# Autodesk Inventor assembly: LR_05
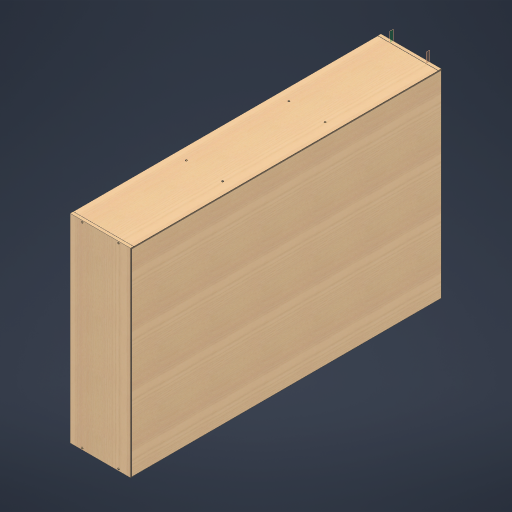
[picture p0: Inventor's stored thumbnail of the model, 512x512]
Saved by Autodesk Inventor 2024.3 (Build 283343000, 343)
## iProperties
Created: 2013-04-03
Part Number: LR_05
Document SubType Name: Assembly
Designer: User
Description: Rack
Author: User
## Documents named in this file (15)
- C:\W4INV 2024 Design\PROJECTS\Living Room\Rack\LR_05.iam
- C:\W4INV 2024 Design\PROJECTS\Samples\Living Room\Rack\LR_0502.ipt
- C:\W4INV 2024 Design\PROJECTS\Samples\Living Room\Rack\LR_0503.ipt
- C:\W4INV 2024 Design\PROJECTS\Samples\Living Room\Rack\LR_0508.ipt
- C:\W4INV 2024 Design\PROJECTS\Samples\Living Room\Rack\LR_0501.ipt
- C:\W4INV 2024 Design\PROJECTS\Samples\Living Room\Rack\LR_0506.ipt
- C:\W4INV 2024 Design\PROJECTS\Samples\Living Room\Rack\LR_0507.ipt
- C:\W4INV 2024 Design\PROJECTS\Samples\Living Room\Rack\LR_0504.ipt
- C:\W4INV 2024 Design\PROJECTS\Samples\Living Room\Rack\LR_0505.ipt
- C:\W4INV 2024 Design\PROJECTS\Samples\Living Room\Rack\SkeletonLR_0500.ipt
- G:\DESIGN\W4I 2014 EN\2013 COMPONENTS LIBRARY\01 CONNECTORS\01 CONFIRMAT\CONFIRMAT & HOLE & CAP.iam
- C:\W4INV 2023 Design\LIBRARY\Holders\Shelf holder D5.ipt
- C:\W4INV 2024 Design\_LIBRARY\Holders\Shelf holder D5\Shelf support D5 L16 HOL 3 CAP ON.ipt
- C:\W4INV 2024 Design\_LIBRARY\Fixed joints\Confirmat\CONFIRMAT\Confirmat L50 & Cap D10 NB T18 PB T 18.ipt
- C:\W4INV 2023 Design\LIBRARY\Fixed joints\Confirmat\CONFIRMAT.ipt
## Components (53 placed, 10 different names)
1. LR_0502-Right Side:2 — Nestled Board Plane:2, Nestled Board Plane:4, Nestled Board Plane:6, Nestled Board Plane:8
2. LR_0503-Left Side:2 — Flush:1, Flush:2, Mate:30, Mate:36, Nestled Board Plane:1, Nestled Board Plane:3, Nestled Board Plane:5, Nestled Board Plane:7
3. LR_0508-Top:2 — Pillar Board Side Plane:1, Pillar Board Side Plane:2, Pillar Board Side Plane:5, Pillar Board Side Plane:6, Nestled Board Plane:9, Nestled Board Plane:11, Nestled Board Plane:13, Nestled Board Plane:15
4. LR_0501-Bottom:2 — Pillar Board Side Plane:3, Pillar Board Side Plane:4, Pillar Board Side Plane:7, Pillar Board Side Plane:8, Nestled Board Plane:10, Nestled Board Plane:12, Nestled Board Plane:14, Nestled Board Plane:16
5. LR_0506-Vertical partition Left:2 — Mate:33, Mate:39, Pillar Board Side Plane:9, Pillar Board Side Plane:10, Pillar Board Side Plane:13, Pillar Board Side Plane:14
6. LR_0507-Vertical partition Right:2 — Pillar Board Side Plane:11, Pillar Board Side Plane:12, Pillar Board Side Plane:15, Pillar Board Side Plane:16
7. LR_0505-Back:2
8. Confirmat L50 & Cap D10 NB T18 PB T 18:1 — Axis Plane:1, Pillar Board Side Plane:1, Nestled Board Plane:1
9. Confirmat L50 & Cap D10 NB T18 PB T 18:2 — Axis Plane:2, Pillar Board Side Plane:2, Nestled Board Plane:2
10. Confirmat L50 & Cap D10 NB T18 PB T 18:3 — Axis Plane:3, Pillar Board Side Plane:3, Nestled Board Plane:3
11. Confirmat L50 & Cap D10 NB T18 PB T 18:4 — Axis Plane:4, Pillar Board Side Plane:4, Nestled Board Plane:4
12. Confirmat L50 & Cap D10 NB T18 PB T 18:5 — Axis Plane:5, Pillar Board Side Plane:5, Nestled Board Plane:5
13. Confirmat L50 & Cap D10 NB T18 PB T 18:6 — Axis Plane:6, Pillar Board Side Plane:6, Nestled Board Plane:6
14. Confirmat L50 & Cap D10 NB T18 PB T 18:7 — Axis Plane:7, Pillar Board Side Plane:7, Nestled Board Plane:7
15. Confirmat L50 & Cap D10 NB T18 PB T 18:8 — Axis Plane:8, Pillar Board Side Plane:8, Nestled Board Plane:8
16. Confirmat L50 & Cap D10 NB T18 PB T 18:9 — Axis Plane:9, Pillar Board Side Plane:9, Nestled Board Plane:9
17. Confirmat L50 & Cap D10 NB T18 PB T 18:10 — Axis Plane:10, Pillar Board Side Plane:10, Nestled Board Plane:10
18. Confirmat L50 & Cap D10 NB T18 PB T 18:11 — Axis Plane:11, Pillar Board Side Plane:11, Nestled Board Plane:11
19. Confirmat L50 & Cap D10 NB T18 PB T 18:12 — Axis Plane:12, Pillar Board Side Plane:12, Nestled Board Plane:12
20. Confirmat L50 & Cap D10 NB T18 PB T 18:13 — Axis Plane:13, Pillar Board Side Plane:13, Nestled Board Plane:13
21. Confirmat L50 & Cap D10 NB T18 PB T 18:14 — Axis Plane:14, Pillar Board Side Plane:14, Nestled Board Plane:14
22. Confirmat L50 & Cap D10 NB T18 PB T 18:15 — Axis Plane:15, Pillar Board Side Plane:15, Nestled Board Plane:15
23. Confirmat L50 & Cap D10 NB T18 PB T 18:16 — Axis Plane:16, Pillar Board Side Plane:16, Nestled Board Plane:16
24. LR_0504-Shelve:7 — Mate:31, Mate:34, Mate:37, Mate:40
25. Shelf support D5 L16 HOL 3 CAP ON:1 — Mate:29, Mate:30, Mate:31
26. Shelf support D5 L16 HOL 3 CAP ON:2 — Mate:32, Mate:33, Mate:34
27. Shelf support D5 L16 HOL 3 CAP ON:3 — Mate:35, Mate:36, Mate:37
28. Shelf support D5 L16 HOL 3 CAP ON:4 — Mate:38, Mate:39, Mate:40
29. LR_0504-Shelve:8
30. Shelf support D5 L16 HOL 3 CAP ON:5
31. Shelf support D5 L16 HOL 3 CAP ON:10
32. Shelf support D5 L16 HOL 3 CAP ON:15
33. Shelf support D5 L16 HOL 3 CAP ON:20
34. LR_0504-Shelve:9
35. Shelf support D5 L16 HOL 3 CAP ON:6
36. Shelf support D5 L16 HOL 3 CAP ON:11
37. Shelf support D5 L16 HOL 3 CAP ON:16
38. Shelf support D5 L16 HOL 3 CAP ON:21
39. LR_0504-Shelve:10
40. Shelf support D5 L16 HOL 3 CAP ON:7
41. Shelf support D5 L16 HOL 3 CAP ON:12
42. Shelf support D5 L16 HOL 3 CAP ON:17
43. Shelf support D5 L16 HOL 3 CAP ON:22
44. LR_0504-Shelve:11
45. Shelf support D5 L16 HOL 3 CAP ON:8
46. Shelf support D5 L16 HOL 3 CAP ON:13
47. Shelf support D5 L16 HOL 3 CAP ON:18
48. Shelf support D5 L16 HOL 3 CAP ON:23
49. LR_0504-Shelve:12
50. Shelf support D5 L16 HOL 3 CAP ON:9
51. Shelf support D5 L16 HOL 3 CAP ON:14
52. Shelf support D5 L16 HOL 3 CAP ON:19
53. Shelf support D5 L16 HOL 3 CAP ON:24
## Component patterns: (6 elements, first: LR_0504-Shelve:7 + Shelf support D5 L16 HOL 3 CAP ON:1 + Shelf support D5 L16 HOL 3 CAP ON:2 + Shelf support D5 L16 HOL 3 CAP ON:3 + Shelf support D5 L16 HOL 3 CAP ON:4)
## Relationships (62: Mate 44, Flush 18)
- Flush:1 (-70 mm): LR_0503-Left Side:2
- Flush:2 (-70 mm): LR_0503-Left Side:2
- Mate:29: Shelf support D5 L16 HOL 3 CAP ON:1
- Mate:30: LR_0503-Left Side:2 ↔ Shelf support D5 L16 HOL 3 CAP ON:1
- Mate:31 (2.5 mm): LR_0504-Shelve:7 ↔ Shelf support D5 L16 HOL 3 CAP ON:1
- Mate:32: Shelf support D5 L16 HOL 3 CAP ON:2
- Mate:33: LR_0506-Vertical partition Left:2 ↔ Shelf support D5 L16 HOL 3 CAP ON:2
- Mate:34 (2.5 mm): LR_0504-Shelve:7 ↔ Shelf support D5 L16 HOL 3 CAP ON:2
- Mate:35: Shelf support D5 L16 HOL 3 CAP ON:3
- Mate:36: LR_0503-Left Side:2 ↔ Shelf support D5 L16 HOL 3 CAP ON:3
- Mate:37 (2.5 mm): LR_0504-Shelve:7 ↔ Shelf support D5 L16 HOL 3 CAP ON:3
- Mate:38: Shelf support D5 L16 HOL 3 CAP ON:4
- Mate:39: LR_0506-Vertical partition Left:2 ↔ Shelf support D5 L16 HOL 3 CAP ON:4
- Mate:40 (2.5 mm): LR_0504-Shelve:7 ↔ Shelf support D5 L16 HOL 3 CAP ON:4
- Axis Plane:1 [Mate]: Confirmat L50 & Cap D10 NB T18 PB T 18:1
- Pillar Board Side Plane:1 [Mate] (-9 mm): LR_0508-Top:2 ↔ Confirmat L50 & Cap D10 NB T18 PB T 18:1
- Nestled Board Plane:1 [Flush]: LR_0503-Left Side:2 ↔ Confirmat L50 & Cap D10 NB T18 PB T 18:1
- Axis Plane:2 [Mate]: Confirmat L50 & Cap D10 NB T18 PB T 18:2
- Pillar Board Side Plane:2 [Mate] (-9 mm): LR_0508-Top:2 ↔ Confirmat L50 & Cap D10 NB T18 PB T 18:2
- Nestled Board Plane:2 [Flush]: LR_0502-Right Side:2 ↔ Confirmat L50 & Cap D10 NB T18 PB T 18:2
- Axis Plane:3 [Mate]: Confirmat L50 & Cap D10 NB T18 PB T 18:3
- Pillar Board Side Plane:3 [Mate] (-9 mm): LR_0501-Bottom:2 ↔ Confirmat L50 & Cap D10 NB T18 PB T 18:3
- Nestled Board Plane:3 [Flush]: LR_0503-Left Side:2 ↔ Confirmat L50 & Cap D10 NB T18 PB T 18:3
- Axis Plane:4 [Mate]: Confirmat L50 & Cap D10 NB T18 PB T 18:4
- Pillar Board Side Plane:4 [Mate] (-9 mm): LR_0501-Bottom:2 ↔ Confirmat L50 & Cap D10 NB T18 PB T 18:4
- Nestled Board Plane:4 [Flush]: LR_0502-Right Side:2 ↔ Confirmat L50 & Cap D10 NB T18 PB T 18:4
- Axis Plane:5 [Mate]: Confirmat L50 & Cap D10 NB T18 PB T 18:5
- Pillar Board Side Plane:5 [Mate] (-9 mm): LR_0508-Top:2 ↔ Confirmat L50 & Cap D10 NB T18 PB T 18:5
- Nestled Board Plane:5 [Flush]: LR_0503-Left Side:2 ↔ Confirmat L50 & Cap D10 NB T18 PB T 18:5
- Axis Plane:6 [Mate]: Confirmat L50 & Cap D10 NB T18 PB T 18:6
- Pillar Board Side Plane:6 [Mate] (-9 mm): LR_0508-Top:2 ↔ Confirmat L50 & Cap D10 NB T18 PB T 18:6
- Nestled Board Plane:6 [Flush]: LR_0502-Right Side:2 ↔ Confirmat L50 & Cap D10 NB T18 PB T 18:6
- Axis Plane:7 [Mate]: Confirmat L50 & Cap D10 NB T18 PB T 18:7
- Pillar Board Side Plane:7 [Mate] (-9 mm): LR_0501-Bottom:2 ↔ Confirmat L50 & Cap D10 NB T18 PB T 18:7
- Nestled Board Plane:7 [Flush]: LR_0503-Left Side:2 ↔ Confirmat L50 & Cap D10 NB T18 PB T 18:7
- Axis Plane:8 [Mate]: Confirmat L50 & Cap D10 NB T18 PB T 18:8
- Pillar Board Side Plane:8 [Mate] (-9 mm): LR_0501-Bottom:2 ↔ Confirmat L50 & Cap D10 NB T18 PB T 18:8
- Nestled Board Plane:8 [Flush]: LR_0502-Right Side:2 ↔ Confirmat L50 & Cap D10 NB T18 PB T 18:8
- Axis Plane:9 [Mate]: Confirmat L50 & Cap D10 NB T18 PB T 18:9
- Pillar Board Side Plane:9 [Mate] (-9 mm): LR_0506-Vertical partition Left:2 ↔ Confirmat L50 & Cap D10 NB T18 PB T 18:9
- Nestled Board Plane:9 [Flush]: LR_0508-Top:2 ↔ Confirmat L50 & Cap D10 NB T18 PB T 18:9
- Axis Plane:10 [Mate]: Confirmat L50 & Cap D10 NB T18 PB T 18:10
- Pillar Board Side Plane:10 [Mate] (-9 mm): LR_0506-Vertical partition Left:2 ↔ Confirmat L50 & Cap D10 NB T18 PB T 18:10
- Nestled Board Plane:10 [Flush]: LR_0501-Bottom:2 ↔ Confirmat L50 & Cap D10 NB T18 PB T 18:10
- Axis Plane:11 [Mate]: Confirmat L50 & Cap D10 NB T18 PB T 18:11
- Pillar Board Side Plane:11 [Mate] (-9 mm): LR_0507-Vertical partition Right:2 ↔ Confirmat L50 & Cap D10 NB T18 PB T 18:11
- Nestled Board Plane:11 [Flush]: LR_0508-Top:2 ↔ Confirmat L50 & Cap D10 NB T18 PB T 18:11
- Axis Plane:12 [Mate]: Confirmat L50 & Cap D10 NB T18 PB T 18:12
- Pillar Board Side Plane:12 [Mate] (-9 mm): LR_0507-Vertical partition Right:2 ↔ Confirmat L50 & Cap D10 NB T18 PB T 18:12
- Nestled Board Plane:12 [Flush]: LR_0501-Bottom:2 ↔ Confirmat L50 & Cap D10 NB T18 PB T 18:12
- Axis Plane:13 [Mate]: Confirmat L50 & Cap D10 NB T18 PB T 18:13
- Pillar Board Side Plane:13 [Mate] (-9 mm): LR_0506-Vertical partition Left:2 ↔ Confirmat L50 & Cap D10 NB T18 PB T 18:13
- Nestled Board Plane:13 [Flush]: LR_0508-Top:2 ↔ Confirmat L50 & Cap D10 NB T18 PB T 18:13
- Axis Plane:14 [Mate]: Confirmat L50 & Cap D10 NB T18 PB T 18:14
- Pillar Board Side Plane:14 [Mate] (-9 mm): LR_0506-Vertical partition Left:2 ↔ Confirmat L50 & Cap D10 NB T18 PB T 18:14
- Nestled Board Plane:14 [Flush]: LR_0501-Bottom:2 ↔ Confirmat L50 & Cap D10 NB T18 PB T 18:14
- Axis Plane:15 [Mate]: Confirmat L50 & Cap D10 NB T18 PB T 18:15
- Pillar Board Side Plane:15 [Mate] (-9 mm): LR_0507-Vertical partition Right:2 ↔ Confirmat L50 & Cap D10 NB T18 PB T 18:15
- Nestled Board Plane:15 [Flush]: LR_0508-Top:2 ↔ Confirmat L50 & Cap D10 NB T18 PB T 18:15
- Axis Plane:16 [Mate]: Confirmat L50 & Cap D10 NB T18 PB T 18:16
- Pillar Board Side Plane:16 [Mate] (-9 mm): LR_0507-Vertical partition Right:2 ↔ Confirmat L50 & Cap D10 NB T18 PB T 18:16
- Nestled Board Plane:16 [Flush]: LR_0501-Bottom:2 ↔ Confirmat L50 & Cap D10 NB T18 PB T 18:16
## Named parameters: Tarp_Lentynu = 377.33333 mm, Tarp_pertvaru = 594 mm
